# Autodesk Inventor assembly: s-assy-unit-j2-2-gear
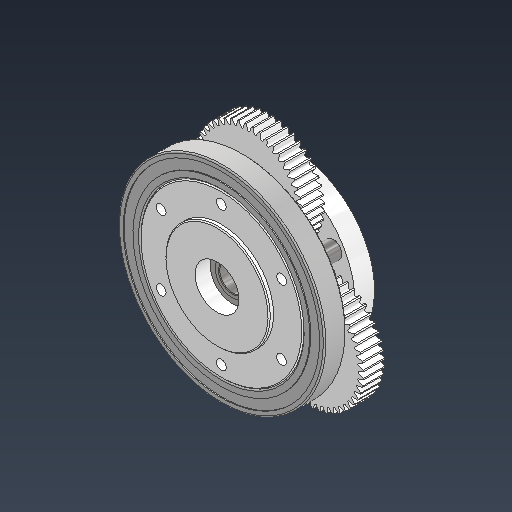
[picture p0: Inventor's stored thumbnail of the model, 512x512]
Saved by Autodesk Inventor 2021 (Build 250183000, 183)
## iProperties
Created: 2021-07-12
Part Number: s-assy-unit-j2-2-gear
Document SubType Name: Assembly
Designer: yuta0
Author: yuta0
## Documents named in this file (10)
- C:\Users\yuta0\Documents\GitHub\catchrobo_hardware\assy-robot\s-assy-unit-j2-2-gear.iam
- C:\Users\yuta0\Documents\GitHub\catchrobo_hardware\assy-robot\base24.ipt
- C:\Users\yuta0\Documents\GitHub\catchrobo_hardware\assy-robot\B6808ZZ.ipt
- C:\Users\yuta0\Documents\GitHub\catchrobo_hardware\assy-robot\ARF-413E.ipt
- C:\Users\yuta0\Documents\GitHub\catchrobo_hardware\assy-robot\s-assy-unit-planet_gear.iam
- C:\Users\yuta0\Documents\GitHub\catchrobo_hardware\assy-robot\CBSTSR4-14.ipt
- C:\Users\yuta0\Documents\GitHub\catchrobo_hardware\assy-robot\carbon_plate11.ipt
- C:\Users\yuta0\Documents\GitHub\catchrobo_hardware\assy-robot\B6815ZZ.ipt
- C:\Users\yuta0\Documents\GitHub\catchrobo_hardware\assy-robot\B6901ZZ.ipt
- C:\Users\yuta0\Documents\GitHub\catchrobo_hardware\assy-robot\base31.ipt
## Components (21 placed, 9 different names)
1. base24:1 — メイト:1, メイト:2, メイト:3, メイト:4, メイト:6, メイト:7, メイト:8
2. B6808ZZ:1 — メイト:1, メイト:2
3. carbon_plate11:1 — メイト:9, メイト:10, メイト:11, メイト:12, メイト:13, メイト:17, メイト:18
4. B6815ZZ:1 — メイト:12, メイト:13, メイト:25
5. base31:1 — メイト:17, メイト:18, メイト:22, メイト:23, メイト:25
6. B6901ZZ:1 — メイト:22, メイト:23
7. unir-spacer1:1 — メイト:3, メイト:4, メイト:5, メイト:9, メイト:10
8. CBSTSR4-14:1 — メイト:7, メイト:8
9. unir-spacer1:2
10. CBSTSR4-14:2
11. unir-spacer1:3
12. CBSTSR4-14:3
13. unir-spacer1:4
14. CBSTSR4-14:4
15. unir-spacer1:5
16. CBSTSR4-14:5
17. unir-spacer1:6
18. CBSTSR4-14:6
19. s-assy-unit-planet_gear:1 [sub-assembly] — メイト:5, メイト:6
20. s-assy-unit-planet_gear:2 [sub-assembly]
21. s-assy-unit-planet_gear:3 [sub-assembly]
## Component patterns: (6 elements, first: unir-spacer1:1 + CBSTSR4-14:1), (3 elements, first: s-assy-unit-planet_gear:1)
## Relationships (18: Mate 18)
- メイト:1 [Mate]: base24:1 ↔ B6808ZZ:1
- メイト:2 [Mate]: base24:1 ↔ B6808ZZ:1
- メイト:3 [Mate]: base24:1 ↔ unir-spacer1:1
- メイト:4 [Mate]: base24:1 ↔ unir-spacer1:1
- メイト:5 [Mate]: unir-spacer1:1 ↔ s-assy-unit-planet_gear:1
- メイト:6 [Mate]: base24:1 ↔ s-assy-unit-planet_gear:1
- メイト:7 [Mate]: base24:1 ↔ CBSTSR4-14:1
- メイト:8 [Mate]: base24:1 ↔ CBSTSR4-14:1
- メイト:9 [Mate]: carbon_plate11:1 ↔ unir-spacer1:1
- メイト:10 [Mate]: carbon_plate11:1 ↔ unir-spacer1:1
- メイト:11 [Mate]: carbon_plate11:1
- メイト:12 [Mate]: carbon_plate11:1 ↔ B6815ZZ:1
- メイト:13 [Mate]: carbon_plate11:1 ↔ B6815ZZ:1
- メイト:17 [Mate]: carbon_plate11:1 ↔ base31:1
- メイト:18 [Mate]: carbon_plate11:1 ↔ base31:1
- メイト:22 [Mate]: base31:1 ↔ B6901ZZ:1
- メイト:23 [Mate]: base31:1 ↔ B6901ZZ:1
- メイト:25 [Mate]: B6815ZZ:1 ↔ base31:1
